# Autodesk Inventor assembly: RobotInforme1
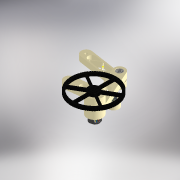
[picture p0: Inventor's stored thumbnail of the model, 180x180]
Saved by Autodesk Inventor 2021 (Build 250183000, 183)
## iProperties
Created: 2024-05-04
Part Number: RobotInforme1
Document SubType Name: Assembly
Designer: Martin
Author: Martin
## Documents named in this file (8)
- C:\Users\ASUS\OneDrive - Universidad de Antioquia\2024-1\Robótica\Proyecto\CAD\op1\RobotInforme1.iam
- C:\Users\ASUS\OneDrive - Universidad de Antioquia\2024-1\Robótica\Proyecto\CAD\37d-gearmotor-19-30-encoder.ipt
- C:\Users\ASUS\OneDrive - Universidad de Antioquia\2024-1\Robótica\Proyecto\CAD\Resorte.ipt
- C:\Users\ASUS\OneDrive - Universidad de Antioquia\2024-1\Robótica\Proyecto\CAD\op1\EslabonCodoTrasero.ipt
- C:\Users\ASUS\OneDrive - Universidad de Antioquia\2024-1\Robótica\Proyecto\CAD\op1\EslabonRodillaCadera.ipt
- C:\Users\ASUS\OneDrive - Universidad de Antioquia\2024-1\Robótica\Proyecto\CAD\op1\EslabonRuedaRodilla.ipt
- C:\Users\ASUS\OneDrive - Universidad de Antioquia\2024-1\Robótica\Proyecto\CAD\op1\Llana.ipt
- C:\Users\ASUS\Documents\Inventor\Content Center Files\R2021\en-US\BS 290 SKF(30)\BS 290 SKF - SKF 608.ipt
## Components (8 placed, 7 different names)
1. 37d-gearmotor-19-30-encoder:1 — Mate:1, Mate:2, Mate:3, Mate:4
2. Resorte:1 — Mate:6, Mate:9
3. EslabonCodoTrasero:1 — Mate:7, Mate:8
4. EslabonRodillaCadera:1 — Mate:9, Mate:10
5. EslabonRuedaRodilla:1 — Mate:1, Mate:2, Mate:3, Mate:5, Mate:6, Mate:7, Mate:8, Mate:10, Mate:11, Mate:12, Mate:13, Mate:14, Mate:15
6. Llana:1 — Mate:4, Mate:5
7. BS 290 SKF 608:1 — Mate:11, Mate:12, Mate:13
8. BS 290 SKF 608:2 — Mate:14, Mate:15
## Relationships (15: Mate 15)
- Mate:1: 37d-gearmotor-19-30-encoder:1 ↔ EslabonRuedaRodilla:1
- Mate:2: 37d-gearmotor-19-30-encoder:1 ↔ EslabonRuedaRodilla:1
- Mate:3: 37d-gearmotor-19-30-encoder:1 ↔ EslabonRuedaRodilla:1
- Mate:4: 37d-gearmotor-19-30-encoder:1 ↔ Llana:1
- Mate:5 (5 mm): EslabonRuedaRodilla:1 ↔ Llana:1
- Mate:6: Resorte:1 ↔ EslabonRuedaRodilla:1
- Mate:7: EslabonCodoTrasero:1 ↔ EslabonRuedaRodilla:1
- Mate:8 (6.7 mm): EslabonCodoTrasero:1 ↔ EslabonRuedaRodilla:1
- Mate:9: Resorte:1 ↔ EslabonRodillaCadera:1
- Mate:10 (40 mm): EslabonRodillaCadera:1 ↔ EslabonRuedaRodilla:1
- Mate:11: EslabonRuedaRodilla:1 ↔ BS 290 SKF 608:1
- Mate:12: EslabonRuedaRodilla:1 ↔ BS 290 SKF 608:1
- Mate:13: EslabonRuedaRodilla:1 ↔ BS 290 SKF 608:1
- Mate:14: EslabonRuedaRodilla:1 ↔ BS 290 SKF 608:2
- Mate:15: EslabonRuedaRodilla:1 ↔ BS 290 SKF 608:2
